# Autodesk Inventor assembly: mg996r 3mm center frame_MIR
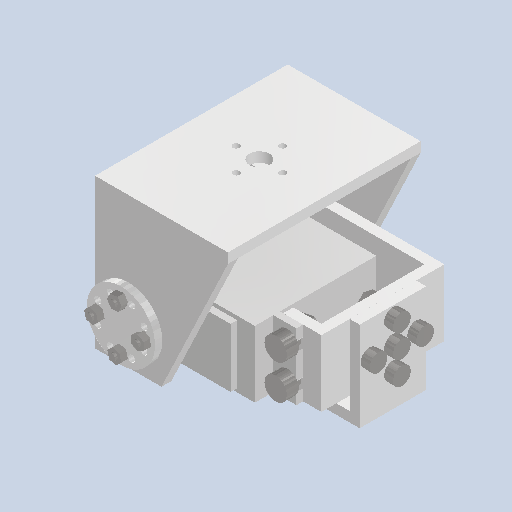
[picture p0: Inventor's stored thumbnail of the model, 512x512]
Saved by Autodesk Inventor 2023 (Build 270158000, 158)
## iProperties
Created: 2022-07-03
Part Number: mg996r 3mm center frame_MIR
Document SubType Name: Assembly
Designer: isamu
Author: isamu
## iProperties of the stored document servo frame mg996 centered_MIR.iam
Created: 2022-07-03
Part Number: servo frame mg996 centered flipped
Description: FreeCAD Model
Document SubType Name: Assembly
Designer: isamu
Authority: Unknown
Sending System: FreeCAD
Preprocessor: Open CASCADE STEP processor 7.5
Title: Open CASCADE Shape Model
Author: Author
## iProperties of the stored document servo frame mg996r009.ipt
Created: 2022-07-03
Part Number: servo frame mg996r009
Material: Generic
Document SubType Name: Modeling
Designer: isamu
Density: 1 g/cm^3
Appearance: Default
Author: isamu
## Documents named in this file (8)
- D:\personal_projects\robot\inventor\mg996r 3mm center frame_MIR.iam
- D:\personal_projects\robot\inventor\base mg996r 3mm with top.iam
- **D:\personal_projects\robot\inventor\mg996r 3mm center frame_MIR.iam*LocalDocs*xAaaaahbaAaaaaaaaAaaaazbl4d*servo frame mg996 centered_MIR.iam
- D:\personal_projects\robot\exports\frames\m2x8.ipt
- D:\personal_projects\robot\exports\frames\m2 nuts.ipt
- D:\personal_projects\robot\exports\frames\m4 nuts.ipt
- **D:\personal_projects\robot\inventor\mg996r 3mm center frame_MIR.iam*LocalDocs*xAaaaqfaaAaaaaaaaAaaaa2ltHh*servo frame mg996r009.ipt
- D:\personal_projects\robot\exports\frames\servo frame mg996 centered_MIR.step
## Components (11 placed, 5 different names)
1. base mg996r 3mm with top:1 [sub-assembly] — Mate:1, Mate:2, Mate:3, Insert:5, Insert:6, Insert:7, Insert:8
2. servo frame mg996 centered_MIR:1 [sub-assembly] — Mate:1, Mate:2, Mate:3, Insert:1, Insert:2, Insert:3, Insert:4, Insert:9
3. m2x8:1 — Insert:2
4. m2x8:2 — Insert:3
5. m2x8:3 — Insert:4
6. m2x8:4 — Insert:1
7. m2 nuts:1 — Insert:5
8. m2 nuts:2 — Insert:7
9. m2 nuts:3 — Insert:8
10. m2 nuts:4 — Insert:6
11. m4 nuts:1 — Insert:9
## Relationships (12: Insert 9, Mate 3)
- Mate:1: base mg996r 3mm with top:1 ↔ servo frame mg996 centered_MIR:1
- Mate:2: base mg996r 3mm with top:1 ↔ servo frame mg996 centered_MIR:1
- Mate:3: base mg996r 3mm with top:1 ↔ servo frame mg996 centered_MIR:1
- Insert:1: servo frame mg996 centered_MIR:1 ↔ m2x8:4
- Insert:2: servo frame mg996 centered_MIR:1 ↔ m2x8:1
- Insert:3: servo frame mg996 centered_MIR:1 ↔ m2x8:2
- Insert:4: servo frame mg996 centered_MIR:1 ↔ m2x8:3
- Insert:5: base mg996r 3mm with top:1 ↔ m2 nuts:1
- Insert:6: base mg996r 3mm with top:1 ↔ m2 nuts:4
- Insert:7: base mg996r 3mm with top:1 ↔ m2 nuts:2
- Insert:8: base mg996r 3mm with top:1 ↔ m2 nuts:3
- Insert:9: servo frame mg996 centered_MIR:1 ↔ m4 nuts:1
